# Autodesk Inventor assembly: Steam Engine 2 inch
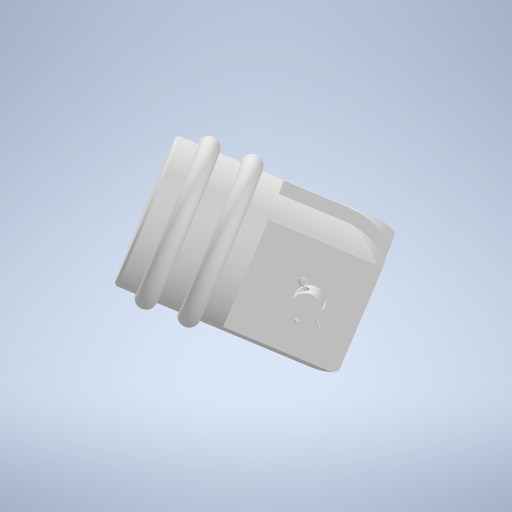
[picture p0: Inventor's stored thumbnail of the model, 512x512]
Saved by Autodesk Inventor 2023 (Build 270158000, 158)
## iProperties
Created: 2022-10-29
Part Number: Steam Engine 2 inch
Document SubType Name: Assembly
Designer: tommy
Author: tommy
## Documents named in this file (5)
- C:\Users\tommy\Documents\Repositories\Steam Engine\2 inch Design V2\Steam Engine 2 inch V2.iam
- C:\Users\tommy\Documents\Repositories\Steam Engine\2 inch Design V2\Piston O Ring.ipt
- C:\Users\tommy\Documents\Repositories\Steam Engine\2 inch Design V2\Piston Head.ipt
- C:\Users\tommy\Documents\Repositories\Steam Engine\2 inch Design V2\Wrist Pin.ipt
- C:\Users\tommy\Documents\Repositories\Steam Engine\2 inch Design V2\Cotter Pin.ipt
## Components (6 placed, 4 different names)
1. Piston Head:1 — Mate:2, Mate:3, Tangent:1, Tangent:2, Mate:11, Mate:14
2. Piston O Ring:1 — Mate:3, Tangent:1
3. Piston O Ring:2 — Mate:2, Tangent:2
4. Wrist Pin:1 — Mate:11, Mate:12, Tangent:4, Mate:13, Tangent:5
5. Cotter Pin:2 — Mate:12, Tangent:4, Mate:14, Angle:1
6. Cotter Pin:3 — Mate:13, Tangent:5, Angle:1
## Relationships (11: Mate 6, Tangent 4, Angle 1)
- Mate:2: Piston Head:1 ↔ Piston O Ring:2
- Mate:3: Piston Head:1 ↔ Piston O Ring:1
- Tangent:1: Piston Head:1 ↔ Piston O Ring:1
- Tangent:2: Piston Head:1 ↔ Piston O Ring:2
- Mate:11: Piston Head:1 ↔ Wrist Pin:1
- Mate:12: Wrist Pin:1 ↔ Cotter Pin:2
- Tangent:4: Wrist Pin:1 ↔ Cotter Pin:2
- Mate:13: Wrist Pin:1 ↔ Cotter Pin:3
- Tangent:5: Wrist Pin:1 ↔ Cotter Pin:3
- Mate:14: Piston Head:1 ↔ Cotter Pin:2
- Angle:1 (0 deg): Cotter Pin:2 ↔ Cotter Pin:3
